# Autodesk Inventor assembly: 조립형상
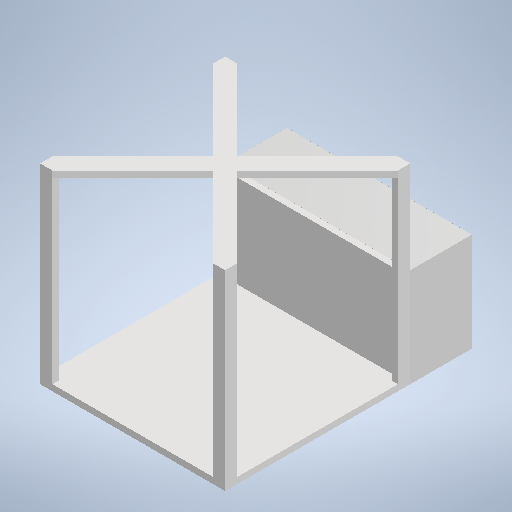
[picture p0: Inventor's stored thumbnail of the model, 512x512]
Saved by Autodesk Inventor 2025 (Build 290162000, 162)
## iProperties
Created: 2024-06-08
Part Number: 조립형상
Document SubType Name: Assembly
Designer: goomi
Author: goomi
## Documents named in this file (4)
- C:\Users\goomi\OneDrive\바탕 화면\기로공\조립형상.iam
- C:\Users\goomi\OneDrive\바탕 화면\기로공\적재부 상판.ipt
- C:\Users\goomi\OneDrive\바탕 화면\기로공\적재부 하판.ipt
- C:\Users\goomi\OneDrive\바탕 화면\기로공\제어부 커버.ipt
## Components (3 placed, 3 different names)
1. 적재부 상판:1 — 강체:1
2. 적재부 하판:1 — 강체:1, 플러쉬:1, 플러쉬:2, 메이트:1, 플러쉬:3
3. 제어부 커버:1 — 플러쉬:1, 플러쉬:2, 메이트:1, 플러쉬:3
## Relationships (5: Flush 3, WeldJoint 1, Mate 1)
- 강체:1 [WeldJoint]: 적재부 상판:1 ↔ 적재부 하판:1
- 플러쉬:1 [Flush]: 적재부 하판:1 ↔ 제어부 커버:1
- 플러쉬:2 [Flush]: 적재부 하판:1 ↔ 제어부 커버:1
- 메이트:1 [Mate]: 적재부 하판:1 ↔ 제어부 커버:1
- 플러쉬:3 [Flush]: 적재부 하판:1 ↔ 제어부 커버:1
